# Autodesk Inventor assembly: 42146-18
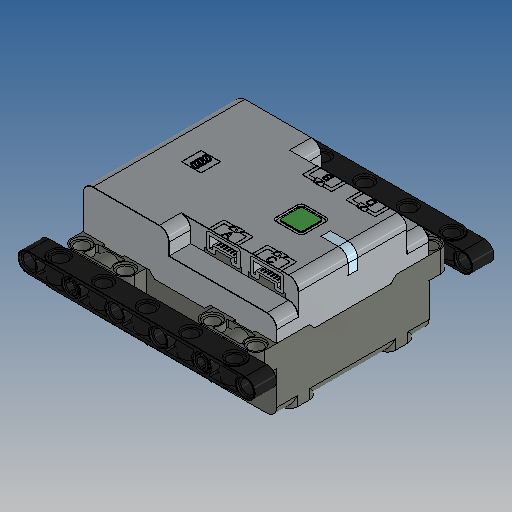
[picture p0: Inventor's stored thumbnail of the model, 512x512]
Saved by Autodesk Inventor 2025 (Build 290162010, 162A)
## iProperties
Created: 2024-11-19
Part Number: 42146-18
Material: Generisch
Document SubType Name: Assembly
Designer: hp.muther
Author: hp.muther
## Documents named in this file (4)
- D:\Inventor\Projekte\Muther\LEGO Technic\LEGO Technik - Raupenkran LR 13000 (42146)\42146-18.iam
- D:\Inventor\Projekte\Muther\LEGO Technic\LEGO Pieces\Lochbalken\73507-Black.ipt
- D:\Inventor\Projekte\Muther\LEGO Technic\LEGO Pieces\Pin's\2780-Black.ipt
- D:\Inventor\Projekte\Muther\LEGO Technic\LEGO Pieces\85824 - HUB.iam
## Components (7 placed, 3 different names)
1. 85824 - HUB:1 [sub-assembly] — Einfügen:6, Passend:2, Einfügen:5, Passend:1
2. 73507-Black:1 — Einfügen:1, Einfügen:2, Einfügen:5
3. 73507-Black:2 — Einfügen:3, Einfügen:4, Einfügen:6
4. 2780-Black:1 — Einfügen:1
5. 2780-Black:2 — Einfügen:2, Passend:1
6. 2780-Black:3 — Einfügen:3
7. 2780-Black:4 — Einfügen:4, Passend:2
## Relationships (8: Insert 6, Mate 2)
- Einfügen:1 [Insert]: 73507-Black:1 ↔ 2780-Black:1
- Einfügen:2 [Insert]: 73507-Black:1 ↔ 2780-Black:2
- Einfügen:3 [Insert]: 73507-Black:2 ↔ 2780-Black:3
- Einfügen:4 [Insert]: 73507-Black:2 ↔ 2780-Black:4
- Einfügen:5 [Insert]: 85824 - HUB:1 ↔ 73507-Black:1
- Passend:1 [Mate]: 85824 - HUB:1 ↔ 2780-Black:2
- Einfügen:6 [Insert]: 85824 - HUB:1 ↔ 73507-Black:2
- Passend:2 [Mate]: 85824 - HUB:1 ↔ 2780-Black:4
